# Autodesk Inventor assembly: motor assembly_MIR
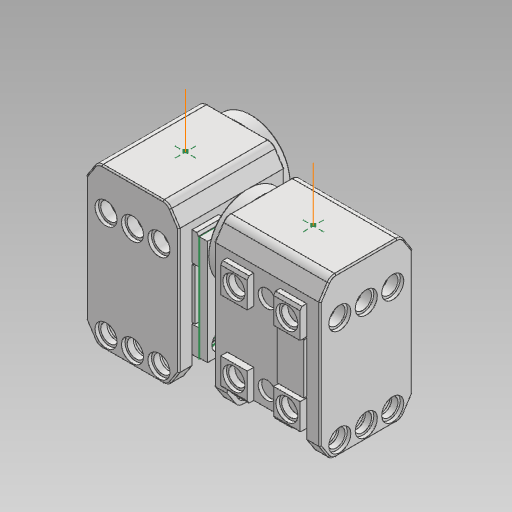
[picture p0: Inventor's stored thumbnail of the model, 512x512]
Saved by Autodesk Inventor 2021 (Build 250183000, 183)
## iProperties
Created: 2020-11-15
Part Number: motor assembly_MIR
Document SubType Name: Assembly
Designer: Kanenas
Mass: 33.2665 g
Surface Area: 117.108 cm^2
Volume: 33.2665 cm^3
Density: 1 g/cm^3
Author: Paco
## Documents named in this file (3)
- C:\Users\Kanenas\Desktop\IISRD_CAD_V\IISRD_V_v1\motor assembly_MIR.iam
- C:\Users\Kanenas\Desktop\IISRD_CAD_V\XL320XL-320_MIR1.ipt
- C:\Users\Kanenas\Desktop\IISRD_CAD_V\IISRD_V_v1\XL_XL_interface_MIR.ipt
## Components (3 placed, 2 different names)
1. XL320XL-320_MIR1:1 — Mate:3, Mate:2, Mate:1
2. XL_XL_interface_MIR:1 — Mate:3, Mate:2, Mate:1, Mate:6, Mate:5, Mate:4
3. XL320XL-320_MIR1:2 — Mate:6, Mate:5, Mate:4
## Relationships (6: Mate 6)
- Mate:3: XL320XL-320_MIR1:1 ↔ XL_XL_interface_MIR:1
- Mate:2: XL320XL-320_MIR1:1 ↔ XL_XL_interface_MIR:1
- Mate:1: XL320XL-320_MIR1:1 ↔ XL_XL_interface_MIR:1
- Mate:6: XL_XL_interface_MIR:1 ↔ XL320XL-320_MIR1:2
- Mate:5: XL_XL_interface_MIR:1 ↔ XL320XL-320_MIR1:2
- Mate:4: XL_XL_interface_MIR:1 ↔ XL320XL-320_MIR1:2
